# Autodesk Inventor assembly: SurubM4x35
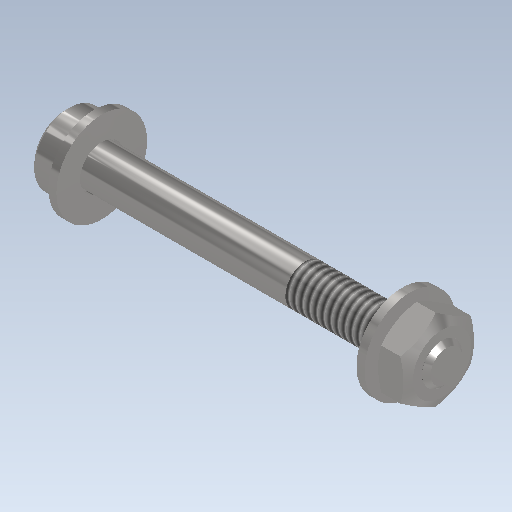
[picture p0: Inventor's stored thumbnail of the model, 512x512]
Saved by Autodesk Inventor 2020 (Build 240168000, 168)
## iProperties
Created: 2021-02-22
Part Number: SurubM4x35
Document SubType Name: Assembly
Designer: Iulian Bors
Mass: 5.53033 g
Surface Area: 10.1799 cm^2
Volume: 0.7045 cm^3
Density: 7.85 g/cm^3
Author: Iulian Bors
## Documents named in this file (4)
- Z:\I.A.B\Proiecte\0008 I.A.B 3D 2.1 Imprimanta aracet Metal\10 Mecanic\SurubM4x35.iam
- Z:\I.A.B\Proiecte\0008 I.A.B 3D 2.1 Imprimanta aracet Metal\10 Mecanic\0008-10-2001 DIN 934 - M4 x 0.7.ipt
- Z:\I.A.B\Proiecte\0008 I.A.B 3D 2.1 Imprimanta aracet Metal\10 Mecanic\0008-10-2002 DIN 125 - A 4.3.ipt
- Z:\I.A.B\Proiecte\0008 I.A.B 3D 2.1 Imprimanta aracet Metal\10 Mecanic\0008-10-2003DIN 6912 - M4 x 35.ipt
## Components (4 placed, 3 different names)
1. 0008-10-2001 DIN 934 - M4 x 0.7.ipt:1 — Insert:2, Insert:4
2. 0008-10-2002 DIN 125 - A 4.3.ipt:2 — Insert:2
3. 0008-10-2002 DIN 125 - A 4.3.ipt:3 — Insert:3
4. 0008-10-2003DIN 6912 - M4 x 35.ipt:4 — Insert:3, Insert:4
## Relationships (3: Insert 3)
- Insert:2: 0008-10-2001 DIN 934 - M4 x 0.7.ipt:1 ↔ 0008-10-2002 DIN 125 - A 4.3.ipt:2
- Insert:3: 0008-10-2002 DIN 125 - A 4.3.ipt:3 ↔ 0008-10-2003DIN 6912 - M4 x 35.ipt:4
- Insert:4: 0008-10-2001 DIN 934 - M4 x 0.7.ipt:1 ↔ 0008-10-2003DIN 6912 - M4 x 35.ipt:4
